# Autodesk Inventor assembly: BD_test
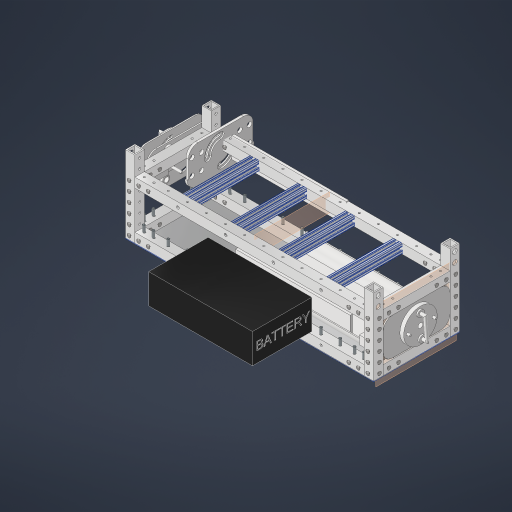
[picture p0: Inventor's stored thumbnail of the model, 512x512]
Saved by Autodesk Inventor 2024 (Build 280153000, 153)
## iProperties
Created: 2024-01-25
Part Number: BD_test
Document SubType Name: Assembly
Designer: seene
Author: seene
## Documents named in this file (6)
- C:\Users\calvi\OneDrive\Robocup Rescue\Chassis\Battery Drawer\BD_test.iam
- C:\Users\calvi\OneDrive\Robocup Rescue\Chassis\Frame\Centerpiece with DTconnector.iam
- Centerpiece.iam
- C:\Users\calvi\OneDrive\Robocup Rescue\Chassis\Battery Drawer\BatteryDrawer.iam
- C:\Users\calvi\OneDrive\Robocup Rescue\Chassis\Battery Drawer\Assembly.iam
- C:\Users\calvi\OneDrive\Robocup Rescue\Chassis\Battery Drawer\Sheet_Assembly.iam
## Components (4 placed, 4 different names)
1. Centerpiece:1 [sub-assembly] — Mate:1, Flush:1, Flush:2, Mate:2, Mate:3, Slider:1, Flush:3
2. BatteryDrawer:1 [sub-assembly] — Mate:1, Flush:1
3. Assembly:1 [sub-assembly] — Flush:2, Mate:2, Mate:3
4. Sheet_Assembly:1 [sub-assembly] — Slider:1, Flush:3
## Relationships (7: Mate 3, Flush 3, TranslationJoint 1)
- Mate:1: Centerpiece:1 ↔ BatteryDrawer:1
- Flush:1: Centerpiece:1 ↔ BatteryDrawer:1
- Flush:2: Centerpiece:1 ↔ Assembly:1
- Mate:2: Centerpiece:1 ↔ Assembly:1
- Mate:3: Centerpiece:1 ↔ Assembly:1
- Slider:1 [TranslationJoint]: Centerpiece:1 ↔ Sheet_Assembly:1
- Flush:3: Centerpiece:1 ↔ Sheet_Assembly:1
